# Autodesk Inventor assembly: 1426_Mitoiu.Bianca-Maria_Ansamblu
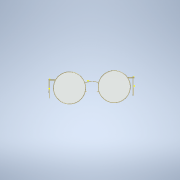
[picture p0: Inventor's stored thumbnail of the model, 180x180]
Saved by Autodesk Inventor 2020 (Build 240168000, 168)
## iProperties
Created: 2020-01-05
Part Number: 1426_Mitoiu.Bianca-Maria_Ansamblu
Document SubType Name: Assembly
Designer: Bianca
Mass: 13.4124 g
Surface Area: 112.147 cm^2
Volume: 3.72637 cm^3
Density: 3.5993 g/cm^3
Author: Bianca
## Documents named in this file (14)
- C:\Users\Bianca\Desktop\ochelari\1426_Mitoiu.Bianca-Maria_Ansamblu.iam
- C:\Users\Bianca\Desktop\ochelari\1426_Mitoiu.Bianca-Maria_Piesa1.ipt
- C:\Users\Bianca\Desktop\ochelari\1426_Mitoiu.Bianca-Maria_piesa2.ipt
- C:\Users\Bianca\Desktop\ochelari\1426_Mitoiu.Bianca-Maria_piesa2_MIR.ipt
- C:\Users\Bianca\Desktop\ochelari\1426_Mitoiu.Bianca-Maria_Piesa3.ipt
- C:\Users\Bianca\Desktop\ochelari\1426_Mitoiu.Bianca-Maria_Piesa3_MIR.ipt
- C:\Users\Bianca\Desktop\ochelari\1426_Mitoiu.Bianca-Maria_Piesa4.ipt
- C:\Users\Bianca\Desktop\ochelari\1426_Mitoiu.Bianca-Maria_Piesa4_MIR.ipt
- C:\Users\Bianca\Desktop\ochelari\1426_Mitoiu.Bianca-Maria_Ansamblu\AIP\FEA\d40w59b8g.fins
- C:\Users\Bianca\Desktop\ochelari\1426_Mitoiu.Bianca-Maria_Ansamblu\AIP\FEA\d40w59b8g.fsat
- C:\Users\Bianca\Desktop\ochelari\1426_Mitoiu.Bianca-Maria_Ansamblu\AIP\FEA\d40w59b8g.ftes
- C:\Users\Bianca\Desktop\ochelari\1426_Mitoiu.Bianca-Maria_Ansamblu\AIP\FEA\d40w59b8g.fwiz
- C:\Users\Bianca\Desktop\ochelari\1426_Mitoiu.Bianca-Maria_Ansamblu\AIP\FEA\d40w59ba8.fmsh
- C:\Users\Bianca\Desktop\ochelari\1426_Mitoiu.Bianca-Maria_Ansamblu\AIP\FEA\d40w59ba9.fres
## Components (7 placed, 7 different names)
1. 1426_Mitoiu.Bianca-Maria_Piesa1:1 — Insert:1, Insert:2, Angle:1, Angle:2, Insert:3, Insert:4, Insert:5, Insert:6
2. 1426_Mitoiu.Bianca-Maria_piesa2:1 — Insert:1, Angle:2
3. 1426_Mitoiu.Bianca-Maria_piesa2_MIR:1 — Insert:2, Angle:1
4. 1426_Mitoiu.Bianca-Maria_Piesa3:1 — Insert:3
5. 1426_Mitoiu.Bianca-Maria_Piesa3_MIR:1 — Insert:4
6. 1426_Mitoiu.Bianca-Maria_Piesa4:1 — Insert:5
7. 1426_Mitoiu.Bianca-Maria_Piesa4_MIR:1 — Insert:6
## Relationships (8: Insert 6, Angle 2)
- Insert:1: 1426_Mitoiu.Bianca-Maria_Piesa1:1 ↔ 1426_Mitoiu.Bianca-Maria_piesa2:1
- Insert:2: 1426_Mitoiu.Bianca-Maria_Piesa1:1 ↔ 1426_Mitoiu.Bianca-Maria_piesa2_MIR:1
- Angle:1 (0 deg): 1426_Mitoiu.Bianca-Maria_Piesa1:1 ↔ 1426_Mitoiu.Bianca-Maria_piesa2_MIR:1
- Angle:2 (180 deg): 1426_Mitoiu.Bianca-Maria_Piesa1:1 ↔ 1426_Mitoiu.Bianca-Maria_piesa2:1
- Insert:3: 1426_Mitoiu.Bianca-Maria_Piesa1:1 ↔ 1426_Mitoiu.Bianca-Maria_Piesa3:1
- Insert:4: 1426_Mitoiu.Bianca-Maria_Piesa1:1 ↔ 1426_Mitoiu.Bianca-Maria_Piesa3_MIR:1
- Insert:5: 1426_Mitoiu.Bianca-Maria_Piesa1:1 ↔ 1426_Mitoiu.Bianca-Maria_Piesa4:1
- Insert:6: 1426_Mitoiu.Bianca-Maria_Piesa1:1 ↔ 1426_Mitoiu.Bianca-Maria_Piesa4_MIR:1
## Named parameters: sa_0 = -456.999, sa_1 = 76.6697, sa_2 = -187.812
note: some values were not read from the file. Shown as the stored number, unit unknown: "sa_0", "sa_1", "sa_2".
